# Autodesk Inventor assembly: GPA60GT2060-B-NK10
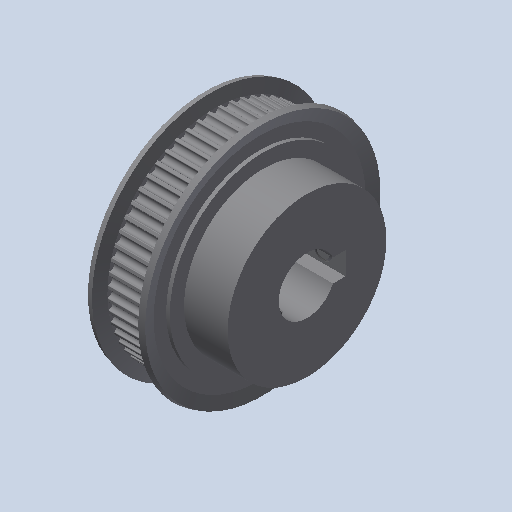
[picture p0: Inventor's stored thumbnail of the model, 512x512]
Saved by Autodesk Inventor 2023 (Build 270158000, 158)
## iProperties
Created: 2022-10-04
Part Number: GPA60GT2060-B-NK10
Catalog Web Link: www.cadenas.de
Description: GPA_GT2040, GPA_GT2060, GPA_GT2090, KGPA_GT2040, KGPA_GT2060, KGPA_GT2090, KGPK_GT2040, KGPK_GT2060, KGPK_GT2090-High Torque Timing Pulleys 2GT Type
Vendor: MISUMI
Document SubType Name: Assembly
Designer: psAdmin
Manufacturer: MISUMI
Mass: 14.444 g
Surface Area: 63.4493 cm^2
Volume: 14.444 cm^3
Density: 1 g/cm^3
Category: PARTsolutions
Company: MISUMI
PSOL_IDENT_0: {$CADENAS_DATA/23d-libs/misumi/metric/51_timing_pulleys/gpa_gt2_asmtab.prj},488 {VTYP=3D},{STYP=ASST
PSOL_IDENT_1: AB},{NB=GPA60GT2060-B-NK10},{LINA=GPA60GT2060-B-NK10},{NN=GPA_GT2040, GPA_GT2060, GPA_GT2090, KGPA_G
PSOL_IDENT_2: T2040, KGPA_GT2060, KGPA_GT2090, KGPK_GT2040, KGPK_GT2060, KGPK_GT2090},{DATE=25.04.2022 01:22:58},{
PSOL_IDENT_3: GEOMDATE=22.12.2021 00:12:27},{VERSION=},{LINEID=190},{WBVAR=MAT,ST,TNW,PS,SBS,DD,Z,J,Q,R,S,T,ALT1,A
PSOL_IDENT_4: LT2,M,QSC,QFC,QTC,ALT3,K,KSC,KFC,KTC,ALT4,ZM,ZSC,ZFC,ZTC,ALT5,BC,ALT6,ALT7,ALT8,FC,ALT13,BN},{WBNUME
PSOL_IDENT_5: RIC=DD,Z,J,Q,R,S,T,QSC,QFC,QTC,K,KSC,KFC,KTC,ZSC,ZFC,ZTC,BC,FC,BN}  {NB=GPA60GT2060-B-NK10},{LINA=GP
PSOL_IDENT_6: A60GT2060-B-NK10},{KT=DUMMY},{PN=GPA60GT2060-B-NK10},{TYPE=GPA},{MAT=AA},{ST=CA},{NT=60},{TNW=GT2060
PSOL_IDENT_7: },{BW=6},{A=7.0},{W=10.3},{L=18.0},{PS=B},{PSA= 'A','B' },{SBS=NK},{SBSALG= 'H','Round Hole','P','Ro
PSOL_IDENT_8: und Hole+Tap','N','New JIS Keywayed Bore + Tap (Standard)','NK','New JIS Keywayed Bore + Tap (keyway
PSOL_IDENT_9: width 4.0mm, height 1.8mm)','V','Stepped Hole','F','Stepped Hole (Counterbore holes on the boss sid
PSOL_IDENT_10: e)' },{DD=10.00},{DDALG=[10:10/1]},{DDHA=[8:29/1]},{DDHB=[8:24/1]},{DDPA=[8:22/1]},{DDPB=[8:22/1]},{
PSOL_IDENT_11: DDNA=8,10,11,12,13,14,15,16,17,18,19},{DDNB=8,10,11,12,13,14},{DDNKA=[10:10/1]},{DDNKB=[10:10/1]},{D
PSOL_IDENT_12: DVA=[8:27/1]},{DDVFB=[8:22/1]},{DDYA=[8:27/1]},{Z=0},{ZALG=0},{ZMIN=12},{ZAMAX=29},{ZBMAX=24},{J=0.0
PSOL_IDENT_13: },{JALG=0},{JMAX=16},{Q=0},{R=0},{QRALG=0},{QRMIN=12},{QRMAX=29},{S=0.0},{SALG=0},{SMAX=4.300},{T=0.
PSOL_IDENT_14: 0},{TALG=0},{TMAX=5.000},{PD=38.20},{OD=37.69},{D=28},{DE=28},{DDZ=10},{F=42},{E=33},{BB=4},{TT=1.8}
PSOL_IDENT_15: ,{M1=4},{AC=M4x3},{ALT1=},{ALT1A= '','w/o Set Screw Angle','-KC90','with KC90 (Set Screw Angle)' },{
PSOL_IDENT_16: ANG=120},{ALT2=},{ALT2A= '','w/o Side Tapped Hole','-QTC','with QTC (3 Places Side Tapped Hole)' },{
PSOL_IDENT_17: M=N/A},{MALG= 'N/A' },{MM=0.000},{MPHD=0.000},{MA= 'N/A' },{MSA= 'N/A' },{QSC=0.0},{QSCA=0},{QFC=0.0
PSOL_IDENT_18: },{QFCA=0},{QTC=0.0},{QTCA=0},{QPCDMIN=14},{QPCDMINALG=14},{QPCDMAX=24},{ALT2PN=},{ALT3=},{ALT3A= ''
PSOL_IDENT_19: ,'w/o Side Through Hole','-KTC','with KTC (3 Places Side Through Hole)' },{K=0.0},{KA=0},{KAMIN=4},{
PSOL_IDENT_20: KAMAX=5},{KSMAX=5},{KSC=0.0},{KSCA=0},{KFC=0.0},{KFCA=0},{KTC=0.0},{KTCA=0},{KSCMIN=14.000},{KPCDMIN=
PSOL_IDENT_21: 14.000},{KPCDMINALG=18.000},{KPCDMAX=24.000},{ALT3PN=},{ALT4=},{ALT4ALG= '','w/o Side Counterbored','
PSOL_IDENT_22: ZTC','with ZTC (3 Places Side Counterbored)' },{ALT4MIN=20.500},{ALT4MAX=20.500},{ZM=N/A},{ZMALG= 'N
PSOL_IDENT_23: /A' },{ZMFTALG= 'N/A' },{ZMSALG= 'N/A' },{ZMDD1=0.0},{ZMDD2=0.0},{ZMHH=0.0},{ZSC=0.0},{ZSCALG=[0]},{
PSOL_IDENT_24: ZFC=0.0},{ZFCALG=[0]},{ZTC=0.0},{ZTCALG=[0]},{ZPCDMIN=0.000},{ZPCDMINALG=0.000},{ZPCDMAX=24.000},{AL
PSOL_IDENT_25: T4PN=},{ALT5=},{ALT5ALG= '','w/o BC (Boss Cut)','-BC','with BC (Boss Cut)' },{ALT5PN=},{BC=0.0},{BCA
PSOL_IDENT_26: LG=0},{BCMIN=7.000},{BCMAX=7.700},{ALT6=},{ALT7=},{ALT7ALG= '','w/o Flange Attached on One Side Only'
PSOL_IDENT_27: ,'-RFC','with RFC (Flange Attached on The Boss Side Only)','-LFC','with LFC (Flange Attached on The
PSOL_IDENT_28: Opposite Side Only)' },{ALT8=},{ALT8ALG='','w/o FC (Flange Cut)','-FC','with FC (Flange Cut)'},{ALT8
PSOL_IDENT_29: PN=},{FC=0.0},{FCA=0},{ODAINT=41.000},{FCMIN=39},{FCMAX=40},{WLBC=18},{SL=6.8},{SL2=5},{KTT=5},{KYY=
PSOL_IDENT_30: 7.2},{TAP=0},{PPATH=gpa__gt2/gpa_gt2_asmtpl.prj},{MATALG= 'AA','Aluminum Alloy 2000 series' , '6000'
PSOL_IDENT_31: ,'6000 Series Aluminum Alloy' },{ALT13=},{BN=0.000},{STALG= 'CA','Clear Anodize' },{BNMIN=8.200},{BN
PSOL_IDENT_32: MAX=17.700},{ALT13ALG= '','w/o BN (Hub Lengthening)','BN','with BN (Hub Lengthening)' },{BNALG=0},{B
PSOL_IDENT_33: NPN=}
NB: GPA60GT2060-B-NK10
NN: GPA_GT2040, GPA_GT2060, GPA_GT2090, KGPA_GT2040, KGPA_GT2060, KGPA_GT2090, KGPK_GT2040, KGPK_GT2060, KGPK_GT2090
NT: 60
NBSYN: $PN.
LINA: GPA60GT2060-B-NK10
CATALOG: Misumi
PN: GPA60GT2060-B-NK10
MAT: Aluminum Alloy 2000 series
ST: Clear Anodize
TNW: GT2060
A: 7
W: 10.3
L: 18
PS: B
SBS: New JIS Keywayed Bore + Tap (keyway width 4.0mm, height 1.8mm)
DD: 10
Z: 0
J: 0
Q: 0
R: 0
S: 0
T: 0
PD: 38.2
OD: 37.69
D: 28
F: 42
E: 33
AC: M4x3
ALT1: w/o Set Screw Angle
ALT2: w/o Side Tapped Hole
M: N/A
QSC: 0
QFC: 0
QTC: 0
ALT3: w/o Side Through Hole
K: 0
KSC: 0
KFC: 0
KTC: 0
ALT4: w/o Side Counterbored
ZM: N/A
ZMDD1: 0
ZMDD2: 0
ZMHH: 0
ZSC: 0
ZFC: 0
ZTC: 0
ALT5: w/o BC (Boss Cut)
BC: 0
ALT6: w/o Flange not Attached
ALT7: w/o Flange Attached on One Side Only
ALT8: w/o FC (Flange Cut)
FC: 0
ALT13: w/o BN (Hub Lengthening)
BN: 0
SUPPLIER: MISUMI
ARTICLENO: GPA60GT2060-B-NK10
BOMINFO: GPA60GT2060-B-NK10
CREATOR: CADENAS GmbH
Title: GPA60GT2060-B-NK10
Author: Cadenas PARTsolutions
Comments: High Torque Timing Pulleys 2GT Type
## Documents named in this file (3)
- C:\Users\Charles Kelly\Documents\Inventor\Robtooc\Apparatus\THE ARM\Hardware\GPA60GT2060-B-NK10.iam
- C:\Users\Charles Kelly\Documents\Inventor\Robtooc\Apparatus\THE ARM\Hardware\GPA60GT2060-B-NK10_b.ipt
- C:\Users\Charles Kelly\Documents\Inventor\Robtooc\Apparatus\THE ARM\Hardware\SET-SCREW4-3.ipt
## Components (3 placed, 2 different names)
1. GPA60GT2060-B-NK10_b:1 — to_screw_B1_Z@1 <-> CP_Z@2, to_screw_B2_Z@1 <-> CP_Z@3
2. SET-SCREW4-3:1 — to_screw_B1_Z@1 <-> CP_Z@2
3. SET-SCREW4-3:2 — to_screw_B2_Z@1 <-> CP_Z@3
## Relationships (2: Mate 2)
- to_screw_B1_Z@1 <-> CP_Z@2 [Mate]: GPA60GT2060-B-NK10_b:1 ↔ SET-SCREW4-3:1
- to_screw_B2_Z@1 <-> CP_Z@3 [Mate]: GPA60GT2060-B-NK10_b:1 ↔ SET-SCREW4-3:2
